# Autodesk Inventor assembly: CNC-FullAssembly
(part 2 of 3)
404. 91274A125-M5x8mm:5
405. 91274A125-M5x8mm:6
406. 91274A125-M5x8mm:7 — Mate:82, Mate:83
407. 91274A125-M5x8mm:8
408. 91274A125-M5x8mm:9
409. 91274A125-M5x8mm:13 — Mate:84, Mate:85
410. 91274A125-M5x8mm:14
411. 91274A125-M5x8mm:15
412. 91274A125-M5x8mm:16
413. 91274A125-M5x8mm:17
414. 91274A125-M5x8mm:18
415. 91274A125-M5x8mm:19 — Mate:86, Mate:87
416. 91274A125-M5x8mm:20
417. 91274A125-M5x8mm:21
418. 91290A231-M5x15mm:41 — Mate:226, Flush:128
419. 91290A231-M5x15mm:40 — Mate:224, Mate:225, Flush:128
420. 91290A231-M5x15mm:67
421. 91290A231-M5x15mm:68
422. 91290A231-M5x15mm:69
423. 91290A231-M5x15mm:70
424. 91290A231-M5x15mm:71
425. 91290A231-M5x15mm:72
426. 91290A231-M5x15mm:73
427. 91290A231-M5x15mm:74
428. 91290A231-M5x15mm:75
429. 91290A231-M5x15mm:76
430. 91290A231-M5x15mm:77
431. 91290A231-M5x15mm:78
432. 91290A231-M5x15mm:79
433. 91290A231-M5x15mm:80
434. 91290A231-M5x15mm:81 — Mate:314
435. 91290A231-M5x15mm:82 — Mate:313
436. 91290A231-M5x15mm:83 — Mate:292, Flush:148
437. 91290A231-M5x15mm:1 — Mate:288, Mate:289, Flush:148
438. 91290A231-M5x15mm:84
439. 91290A231-M5x15mm:85
440. 91290A231-M5x15mm:86
441. 91290A231-M5x15mm:87
442. 91290A231-M5x15mm:88
443. 91290A231-M5x15mm:89
444. 91290A231-M5x15mm:90
445. 91290A231-M5x15mm:91
446. 91290A231-M5x15mm:92
447. 91290A231-M5x15mm:93
448. 91290A231-M5x15mm:94
449. 91290A231-M5x15mm:95
450. 91290A231-M5x15mm:114 — Mate:595, Flush:298
451. 91290A231-M5x15mm:116
452. 91290A231-M5x15mm:117
453. 91290A231-M5x15mm:118
454. 91290A231-M5x15mm:115 — Mate:596, Flush:297, Flush:298
455. 91290A231-M5x15mm:119
456. 91290A231-M5x15mm:120
457. 91290A231-M5x15mm:121
458. 91290A231-M5x15mm:113 — Mate:597, Flush:296, Flush:297
459. 91290A231-M5x15mm:122
460. 91290A231-M5x15mm:123
461. 91290A231-M5x15mm:124
462. 91290A231-M5x15mm:112 — Mate:598, Mate:599, Flush:296
463. 91290A231-M5x15mm:125
464. 91290A231-M5x15mm:126
465. 91290A231-M5x15mm:127
466. 91290A231-M5x15mm:128 — Mate:622, Mate:623
467. 91290A231-M5x15mm:129
468. 91290A231-M5x15mm:130
## Component patterns: (4 elements, first: 91290A231-M5x15mm:20), (4 elements, first: 91290A231-M5x15mm:19), (6 elements, first: 91274A125-M5x8mm:1), (3 elements, first: 91274A125-M5x8mm:7), (6 elements, first: 91274A125-M5x8mm:13), (3 elements, first: 91274A125-M5x8mm:19), (9 elements, first: 91290A231-M5x15mm:41 + 91290A231-M5x15mm:40), (7 elements, first: 91290A231-M5x15mm:83 + 91290A231-M5x15mm:1), (4 elements, first: 91290A231-M5x15mm:114), (4 elements, first: 91290A231-M5x15mm:115), (4 elements, first: 91290A231-M5x15mm:113), (4 elements, first: 91290A231-M5x15mm:112), (3 elements, first: 91290A231-M5x15mm:128)
## Relationships (920: Mate 599, Flush 280, Angle 26, Tangent 14, Symmetry 1)
- Mate:1 (-20 mm): 40x40x500mm-Extrusion:1
- Mate:2 (-20 mm): 40x40x500mm-Extrusion:1
- Flush:1 (-250 mm): 40x40x500mm-Extrusion:1
- Flush:2: 40x40x500mm-Extrusion:1 ↔ 40x40x500mm-Extrusion:2
- Flush:3: 40x40x500mm-Extrusion:1 ↔ 40x40x500mm-Extrusion:2
- Mate:3: SFU1605-BallScrewNut:1 ↔ DSG16H-BallScrewFixtureBlock:1
- Mate:4: SFU1605-BallScrewNut:1 ↔ DSG16H-BallScrewFixtureBlock:1
- Mate:5: SFU1605-BallScrewNut:1 ↔ DSG16H-BallScrewFixtureBlock:1
- Angle:1 (0 deg): 40x40x500mm-Extrusion:1 ↔ DSG16H-BallScrewFixtureBlock:1
- Angle:2 (0 deg): 40x40x500mm-Extrusion:2 ↔ BK12-BallScrewStabilizer:1
- Flush:10: HGH20-LinearRailCarriage:1 ↔ HGH20-LinearRailCarriage:3
- Flush:11: HGH20-LinearRailCarriage:1 ↔ HGH20-LinearRailCarriage:4
- Mate:18 (40 mm): HGH20-LinearRailCarriage:1 ↔ HGH20-LinearRailCarriage:4
- Flush:12: HGH20-LinearRailCarriage:2 ↔ HGH20-LinearRailCarriage:3
- Flush:13: HGH20-LinearRailCarriage:2 ↔ HGH20-LinearRailCarriage:4
- Flush:14: DSG16H-BallScrewFixtureBlock:1 ↔ HGH20-LinearRailCarriage:1
- Mate:20: DSG16H-BallScrewFixtureBlock:1 ↔ HGH20-LinearRailCarriage:3
- Mate:21: SFU1605-BallScrewNut:1 ↔ 91274A131_M5x20mm:1
- Mate:22: SFU1605-BallScrewNut:1 ↔ 91274A131_M5x20mm:1
- Mate:23: SFU1605-BallScrewNut:1 ↔ 91274A131_M5x20mm:5
- Mate:24: SFU1605-BallScrewNut:1 ↔ 91274A131_M5x20mm:6
- Mate:25: SFU1605-BallScrewNut:1 ↔ 91274A131_M5x20mm:4
- Mate:26: SFU1605-BallScrewNut:1 ↔ 91274A131_M5x20mm:2
- Mate:27: SFU1605-BallScrewNut:1 ↔ 91274A131_M5x20mm:3
- Flush:15: 91274A131_M5x20mm:2 ↔ 91274A131_M5x20mm:3
- Flush:16: 91274A131_M5x20mm:2 ↔ 91274A131_M5x20mm:4
- Flush:17: 91274A131_M5x20mm:1 ↔ 91274A131_M5x20mm:4
- Flush:18: 91274A131_M5x20mm:1 ↔ 91274A131_M5x20mm:5
- Flush:19: 91274A131_M5x20mm:5 ↔ 91274A131_M5x20mm:6
- Mate:32: Nema23-StepperMotor:1 ↔ MH2025-6.35x10mmCoupler:1
- Angle:3 (0 deg): 40x40x500mm-Extrusion:1 ↔ Nema23-StepperMotor:1
- Mate:33 (2 mm): Nema23-StepperMotor:1 ↔ MH2025-6.35x10mmCoupler:1
- Angle:4 (0 deg): 40x40x500mm-Extrusion:1 ↔ BF12-BallScrewStabilizer2:1
- Mate:39: 40x40x500mm-Extrusion:2 ↔ CNC-000-StructureGusset1:1
- Mate:40: 40x40x500mm-Extrusion:2 ↔ CNC-000-StructureGusset1:1
- Mate:41: 40x40x500mm-Extrusion:2 ↔ CNC-000-StructureGusset1:1
- Mate:42: CNC-000-StructureGusset1:1 ↔ 91290A231-M5x15mm:19
- Mate:43: CNC-000-StructureGusset1:1 ↔ 91290A231-M5x15mm:19
- Mate:44: CNC-000-StructureGusset1:1 ↔ 91290A231-M5x15mm:20
- Mate:45: CNC-000-StructureGusset1:1 ↔ 91290A231-M5x15mm:20
- Flush:20: 40x40x500mm-Extrusion:1 ↔ 20x40x500mm-Extrusion:1
- Flush:21: 40x40x500mm-Extrusion:1 ↔ 20x40x500mm-Extrusion:1
- Flush:22: 40x40x500mm-Extrusion:2 ↔ 20x40x500mm-Extrusion:2
- Flush:23: 40x40x500mm-Extrusion:2 ↔ 20x40x500mm-Extrusion:2
- Mate:48: 40x40x500mm-Extrusion:1 ↔ CNC-001-StructureGusset2:1
- Mate:49: 40x40x500mm-Extrusion:1 ↔ CNC-001-StructureGusset2:1
- Mate:51: CNC-001-StructureGusset2:1 ↔ 91290A231-M5x15mm:27
- Mate:52: CNC-001-StructureGusset2:1 ↔ 91290A231-M5x15mm:27
- Mate:53: CNC-001-StructureGusset2:1 ↔ 91290A231-M5x15mm:30
- Mate:54: CNC-001-StructureGusset2:1 ↔ 91290A231-M5x15mm:28
- Mate:55: CNC-001-StructureGusset2:1 ↔ 91290A231-M5x15mm:29
- Flush:24: 91290A231-M5x15mm:28 ↔ 91290A231-M5x15mm:29
- Flush:25: 91290A231-M5x15mm:27 ↔ 91290A231-M5x15mm:28
- Flush:26: 91290A231-M5x15mm:27 ↔ 91290A231-M5x15mm:30
- Mate:56: BF12-BallScrewStabilizer2:1 ↔ CNC-002-ShimStructureGusset2:1
- Mate:57: BF12-BallScrewStabilizer2:1 ↔ CNC-002-ShimStructureGusset2:1
- Mate:58: BF12-BallScrewStabilizer2:1 ↔ CNC-002-ShimStructureGusset2:1
- Mate:59: Nema23-StepperMotor:1 ↔ 91274A131_M5x20mm:9
- Mate:60: Nema23-StepperMotor:1 ↔ 91274A131_M5x20mm:7
- Mate:61: Nema23-StepperMotor:1 ↔ 91274A131_M5x20mm:10
- Mate:62: Nema23-StepperMotor:1 ↔ 91274A131_M5x20mm:8
- Mate:63: Nema23-StepperMotor:1 ↔ 91274A131_M5x20mm:8
- Flush:27: 91274A131_M5x20mm:8 ↔ 91274A131_M5x20mm:10
- Flush:28: 91274A131_M5x20mm:9 ↔ 91274A131_M5x20mm:10
- Flush:29: 91274A131_M5x20mm:7 ↔ 91274A131_M5x20mm:9
- Mate:64: 91274A131_M5x20mm:9 ↔ 90576A104-M5-NylockNut:1
- Mate:65: CNC-000-StructureGusset1:1 ↔ 90576A104-M5-NylockNut:1
- Mate:66: 91274A131_M5x20mm:10 ↔ 90576A104-M5-NylockNut:2
- Mate:67: 91274A131_M5x20mm:7 ↔ 90576A104-M5-NylockNut:4
- Mate:68: 91274A131_M5x20mm:8 ↔ 90576A104-M5-NylockNut:3
- Flush:30: 90576A104-M5-NylockNut:2 ↔ 90576A104-M5-NylockNut:3
- Flush:31: 90576A104-M5-NylockNut:3 ↔ 90576A104-M5-NylockNut:4
- Flush:32: 90576A104-M5-NylockNut:1 ↔ 90576A104-M5-NylockNut:4
- Mate:75: 20x40x500mm-Extrusion:1 ↔ CNC-003-StructureGusset3:1
- Flush:35 (4.225 mm): 40x40x500mm-Extrusion:1 ↔ CNC-003-StructureGusset3:1
- Flush:36 (-4.225 mm): 20x40x500mm-Extrusion:1 ↔ CNC-003-StructureGusset3:1
- Mate:76: 20x40x500mm-Extrusion:2 ↔ CNC-003-StructureGusset3:2
- Flush:37 (-4.225 mm): 20x40x500mm-Extrusion:2 ↔ CNC-003-StructureGusset3:2
- Flush:38 (4.225 mm): 40x40x500mm-Extrusion:2 ↔ CNC-003-StructureGusset3:2
- Mate:77: CNC-000-StructureGusset1:1 ↔ CNC-004-Nema23Shim:1
- Mate:78: 90576A104-M5-NylockNut:2 ↔ CNC-004-Nema23Shim:1
- Mate:79: CNC-000-StructureGusset1:1 ↔ CNC-004-Nema23Shim:1
- Mate:80: CNC-003-StructureGusset3:1 ↔ 91274A125-M5x8mm:1
- Mate:81: CNC-003-StructureGusset3:1 ↔ 91274A125-M5x8mm:1
- Mate:82: CNC-003-StructureGusset3:1 ↔ 91274A125-M5x8mm:7
- Mate:83: CNC-003-StructureGusset3:1 ↔ 91274A125-M5x8mm:7
- Mate:84: CNC-003-StructureGusset3:2 ↔ 91274A125-M5x8mm:13
- Mate:85: CNC-003-StructureGusset3:2 ↔ 91274A125-M5x8mm:13
- Mate:86: CNC-003-StructureGusset3:2 ↔ 91274A125-M5x8mm:19
- Mate:87: CNC-003-StructureGusset3:2 ↔ 91274A125-M5x8mm:19
- Mate:91: HGH20-LinearRailCarriage:5 ↔ HGR20R-LinearRail500mm:4
- Mate:92: HGH20-LinearRailCarriage:5 ↔ HGR20R-LinearRail500mm:4
- Flush:50: HGR20R-LinearRail500mm:3 ↔ HGR20R-LinearRail500mm:4
- Angle:6 (180 deg): DSG16H-BallScrewFixtureBlock:1 ↔ DSG16H-BallScrewFixtureBlock:2
- Mate:94: DSG16H-BallScrewFixtureBlock:2 ↔ SFU1605-BallScrewNut:2
- Mate:95: DSG16H-BallScrewFixtureBlock:2 ↔ SFU1605-BallScrewNut:2
- Mate:96: DSG16H-BallScrewFixtureBlock:2 ↔ SFU1605-BallScrewNut:2
- Mate:97: DSG16H-BallScrewFixtureBlock:2 ↔ SFU1605-BallScrew500mm:2
- Mate:98: DSG16H-BallScrewFixtureBlock:1 ↔ CNC-005-XAxisMount1:1
- Mate:99: DSG16H-BallScrewFixtureBlock:1 ↔ CNC-005-XAxisMount1:1
- Mate:100: HGH20-LinearRailCarriage:1 ↔ CNC-005-XAxisMount1:1
- Mate:101: CNC-005-XAxisMount1:1 ↔ 91263A832-M5x10mm-Countersink:1
- Flush:53: CNC-005-XAxisMount1:1 ↔ 91263A832-M5x10mm-Countersink:1
- Mate:102: CNC-005-XAxisMount1:1 ↔ 91263A832-M5x10mm-Countersink:3
- Mate:103: CNC-005-XAxisMount1:1 ↔ 91263A832-M5x10mm-Countersink:4
- Mate:104: CNC-005-XAxisMount1:1 ↔ 91263A832-M5x10mm-Countersink:2
- Flush:54: 91263A832-M5x10mm-Countersink:3 ↔ 91263A832-M5x10mm-Countersink:4
- Flush:55: 91263A832-M5x10mm-Countersink:2 ↔ 91263A832-M5x10mm-Countersink:3
- Flush:56: 91263A832-M5x10mm-Countersink:1 ↔ 91263A832-M5x10mm-Countersink:3
- Mate:105: CNC-005-XAxisMount1:1 ↔ 91263A832-M5x10mm-Countersink:5
- Mate:106: CNC-005-XAxisMount1:1 ↔ 91263A832-M5x10mm-Countersink:6
- Mate:107: CNC-005-XAxisMount1:1 ↔ 91263A832-M5x10mm-Countersink:8
- Mate:108: CNC-005-XAxisMount1:1 ↔ 91263A832-M5x10mm-Countersink:7
- Flush:57: CNC-005-XAxisMount1:1 ↔ 91263A832-M5x10mm-Countersink:7
- Flush:58: CNC-005-XAxisMount1:1 ↔ 91263A832-M5x10mm-Countersink:6
- Flush:59: CNC-005-XAxisMount1:1 ↔ 91263A832-M5x10mm-Countersink:5
- Flush:60: CNC-005-XAxisMount1:1 ↔ 91263A832-M5x10mm-Countersink:8
- Mate:109: CNC-005-XAxisMount1:1 ↔ 91263A832-M5x10mm-Countersink:11
- Mate:110: CNC-005-XAxisMount1:1 ↔ 91263A832-M5x10mm-Countersink:12
- Mate:111: CNC-005-XAxisMount1:1 ↔ 91263A832-M5x10mm-Countersink:10
- Mate:112: CNC-005-XAxisMount1:1 ↔ 91263A832-M5x10mm-Countersink:9
- Flush:61: CNC-005-XAxisMount1:1 ↔ 91263A832-M5x10mm-Countersink:10
- Flush:62: 91263A832-M5x10mm-Countersink:9 ↔ 91263A832-M5x10mm-Countersink:10
- Flush:63: CNC-005-XAxisMount1:1 ↔ 91263A832-M5x10mm-Countersink:11
- Flush:64: 91263A832-M5x10mm-Countersink:11 ↔ 91263A832-M5x10mm-Countersink:12
- Mate:113: CNC-005-XAxisMount1:1 ↔ 91263A832-M5x10mm-Countersink:13
- Mate:114: CNC-005-XAxisMount1:1 ↔ 91263A832-M5x10mm-Countersink:16
- Mate:115: CNC-005-XAxisMount1:1 ↔ 91263A832-M5x10mm-Countersink:15
- Mate:116: CNC-005-XAxisMount1:1 ↔ 91263A832-M5x10mm-Countersink:14
- Flush:65: CNC-005-XAxisMount1:1 ↔ 91263A832-M5x10mm-Countersink:13
- Flush:66: CNC-005-XAxisMount1:1 ↔ 91263A832-M5x10mm-Countersink:15
- Flush:67: CNC-005-XAxisMount1:1 ↔ 91263A832-M5x10mm-Countersink:14
- Flush:68: CNC-005-XAxisMount1:1 ↔ 91263A832-M5x10mm-Countersink:16
- Mate:117: CNC-005-XAxisMount1:1 ↔ 91263A832-M5x10mm-Countersink:19
- Mate:118: CNC-005-XAxisMount1:1 ↔ 91263A832-M5x10mm-Countersink:17
- Mate:119: CNC-005-XAxisMount1:1 ↔ 91263A832-M5x10mm-Countersink:18
- Mate:120: CNC-005-XAxisMount1:1 ↔ 91263A832-M5x10mm-Countersink:20
- Flush:69: CNC-005-XAxisMount1:1 ↔ 91263A832-M5x10mm-Countersink:18
- Flush:70: CNC-005-XAxisMount1:1 ↔ 91263A832-M5x10mm-Countersink:20
- Flush:71: CNC-005-XAxisMount1:1 ↔ 91263A832-M5x10mm-Countersink:17
- Flush:72: CNC-005-XAxisMount1:1 ↔ 91263A832-M5x10mm-Countersink:19
- Mate:121: DSG16H-BallScrewFixtureBlock:2 ↔ CNC-006-XAxisMount2:1
- Mate:122: DSG16H-BallScrewFixtureBlock:2 ↔ CNC-006-XAxisMount2:1
- Mate:123: DSG16H-BallScrewFixtureBlock:2 ↔ CNC-006-XAxisMount2:1
- Mate:124: CNC-005-XAxisMount1:1 ↔ CNC-006-XAxisMount2:1
- Angle:7 (0 deg): CNC-005-XAxisMount1:1 ↔ CNC-006-XAxisMount2:1
- Mate:125: HGH20-LinearRailCarriage:7 ↔ CNC-006-XAxisMount2:1
- Mate:126: HGH20-LinearRailCarriage:7 ↔ CNC-006-XAxisMount2:1
- Mate:127: HGH20-LinearRailCarriage:7 ↔ CNC-006-XAxisMount2:1
- Mate:128: HGH20-LinearRailCarriage:6 ↔ CNC-006-XAxisMount2:1
- Mate:129: HGH20-LinearRailCarriage:6 ↔ CNC-006-XAxisMount2:1
- Mate:130: HGH20-LinearRailCarriage:6 ↔ CNC-006-XAxisMount2:1
- Mate:131: HGH20-LinearRailCarriage:5 ↔ CNC-006-XAxisMount2:1
- Mate:132: HGH20-LinearRailCarriage:5 ↔ CNC-006-XAxisMount2:1
- Mate:133: HGH20-LinearRailCarriage:5 ↔ CNC-006-XAxisMount2:1
- Mate:134: HGH20-LinearRailCarriage:8 ↔ CNC-006-XAxisMount2:1
- Mate:135: HGH20-LinearRailCarriage:8 ↔ CNC-006-XAxisMount2:1
- Mate:136: HGH20-LinearRailCarriage:8 ↔ CNC-006-XAxisMount2:1
- Mate:137: HGH20-LinearRailCarriage:8 ↔ HGR20R-LinearRail500mm:3
- Mate:138: HGH20-LinearRailCarriage:8 ↔ HGR20R-LinearRail500mm:3
- Mate:139: SFU1605-BallScrewNut:2 ↔ 91274A131_M5x20mm:11
- Mate:140: SFU1605-BallScrewNut:2 ↔ 91274A131_M5x20mm:11
- Mate:141: SFU1605-BallScrewNut:2 ↔ 91274A131_M5x20mm:14
- Mate:142: SFU1605-BallScrewNut:2 ↔ 91274A131_M5x20mm:16
- Mate:143: SFU1605-BallScrewNut:2 ↔ 91274A131_M5x20mm:15
- Mate:144: SFU1605-BallScrewNut:2 ↔ 91274A131_M5x20mm:13
- Mate:145: SFU1605-BallScrewNut:2 ↔ 91274A131_M5x20mm:12
- Flush:73: 91274A131_M5x20mm:14 ↔ 91274A131_M5x20mm:16
- Flush:74: 91274A131_M5x20mm:11 ↔ 91274A131_M5x20mm:14
- Flush:75: 91274A131_M5x20mm:11 ↔ 91274A131_M5x20mm:15
- Flush:76: 91274A131_M5x20mm:12 ↔ 91274A131_M5x20mm:16
- Flush:77: 91274A131_M5x20mm:12 ↔ 91274A131_M5x20mm:13
- Mate:146: CNC-006-XAxisMount2:1 ↔ 91263A832-M5x10mm-Countersink:22
- Mate:147: CNC-006-XAxisMount2:1 ↔ 91263A832-M5x10mm-Countersink:23
- Mate:148: CNC-006-XAxisMount2:1 ↔ 91263A832-M5x10mm-Countersink:24
- Mate:149: CNC-006-XAxisMount2:1 ↔ 91263A832-M5x10mm-Countersink:21
- Flush:78: CNC-006-XAxisMount2:1 ↔ 91263A832-M5x10mm-Countersink:21
- Flush:79: CNC-006-XAxisMount2:1 ↔ 91263A832-M5x10mm-Countersink:23
- Flush:80: 91263A832-M5x10mm-Countersink:22 ↔ 91263A832-M5x10mm-Countersink:23
- Flush:81: CNC-006-XAxisMount2:1 ↔ 91263A832-M5x10mm-Countersink:24
- Mate:150: CNC-006-XAxisMount2:1 ↔ 91263A832-M5x10mm-Countersink:25
- Mate:151: CNC-006-XAxisMount2:1 ↔ 91263A832-M5x10mm-Countersink:27
- Mate:152: CNC-006-XAxisMount2:1 ↔ 91263A832-M5x10mm-Countersink:28
- Mate:153: CNC-006-XAxisMount2:1 ↔ 91263A832-M5x10mm-Countersink:26
- Flush:82: CNC-006-XAxisMount2:1 ↔ 91263A832-M5x10mm-Countersink:27
- Flush:83: CNC-006-XAxisMount2:1 ↔ 91263A832-M5x10mm-Countersink:26
- Flush:84: CNC-006-XAxisMount2:1 ↔ 91263A832-M5x10mm-Countersink:28
- Flush:85: CNC-006-XAxisMount2:1 ↔ 91263A832-M5x10mm-Countersink:25
- Mate:154: CNC-006-XAxisMount2:1 ↔ 91263A832-M5x10mm-Countersink:31
- Mate:155: CNC-006-XAxisMount2:1 ↔ 91263A832-M5x10mm-Countersink:30
- Mate:156: CNC-006-XAxisMount2:1 ↔ 91263A832-M5x10mm-Countersink:29
- Mate:157: CNC-006-XAxisMount2:1 ↔ 91263A832-M5x10mm-Countersink:32
- Flush:86: CNC-006-XAxisMount2:1 ↔ 91263A832-M5x10mm-Countersink:32
- Flush:87: CNC-006-XAxisMount2:1 ↔ 91263A832-M5x10mm-Countersink:29
- Flush:88: 91263A832-M5x10mm-Countersink:29 ↔ 91263A832-M5x10mm-Countersink:31
- Flush:89: 91263A832-M5x10mm-Countersink:30 ↔ 91263A832-M5x10mm-Countersink:31
- Mate:158: CNC-006-XAxisMount2:1 ↔ 91263A832-M5x10mm-Countersink:35
- Mate:159: CNC-006-XAxisMount2:1 ↔ 91263A832-M5x10mm-Countersink:33
- Mate:160: CNC-006-XAxisMount2:1 ↔ 91263A832-M5x10mm-Countersink:34
- Mate:161: CNC-006-XAxisMount2:1 ↔ 91263A832-M5x10mm-Countersink:36
- Flush:90: CNC-006-XAxisMount2:1 ↔ 91263A832-M5x10mm-Countersink:36
- Flush:91: CNC-006-XAxisMount2:1 ↔ 91263A832-M5x10mm-Countersink:34
- Flush:92: CNC-006-XAxisMount2:1 ↔ 91263A832-M5x10mm-Countersink:35
- Flush:93: CNC-006-XAxisMount2:1 ↔ 91263A832-M5x10mm-Countersink:33
- Mate:162: CNC-006-XAxisMount2:1 ↔ 91263A832-M5x10mm-Countersink:38
- Mate:163: CNC-006-XAxisMount2:1 ↔ 91263A832-M5x10mm-Countersink:39
- Mate:164: CNC-006-XAxisMount2:1 ↔ 91263A832-M5x10mm-Countersink:37
- Mate:165: CNC-006-XAxisMount2:1 ↔ 91263A832-M5x10mm-Countersink:40
- Flush:94: CNC-006-XAxisMount2:1 ↔ 91263A832-M5x10mm-Countersink:40
- Flush:95: CNC-006-XAxisMount2:1 ↔ 91263A832-M5x10mm-Countersink:37
- Flush:96: CNC-006-XAxisMount2:1 ↔ 91263A832-M5x10mm-Countersink:38
- Flush:97: CNC-006-XAxisMount2:1 ↔ 91263A832-M5x10mm-Countersink:39
- Mate:166: CNC-005-XAxisMount1:1 ↔ CNC-006-XAxisMount2:1
- Mate:167: CNC-006-XAxisMount2:1 ↔ 92095A495-M8-18mm-ButtonHead:1
- Mate:168: CNC-006-XAxisMount2:1 ↔ 92095A495-M8-18mm-ButtonHead:2
- Mate:169: CNC-006-XAxisMount2:1 ↔ 92095A495-M8-18mm-ButtonHead:3
- Mate:170: CNC-006-XAxisMount2:1 ↔ 92095A495-M8-18mm-ButtonHead:3
- Flush:98: 92095A495-M8-18mm-ButtonHead:1 ↔ 92095A495-M8-18mm-ButtonHead:3
- Flush:99: 92095A495-M8-18mm-ButtonHead:1 ↔ 92095A495-M8-18mm-ButtonHead:2
- Mate:171: CNC-006-XAxisMount2:1 ↔ 92095A495-M8-18mm-ButtonHead:8
- Flush:100: 92095A495-M8-18mm-ButtonHead:3 ↔ 92095A495-M8-18mm-ButtonHead:8
- Mate:172: CNC-006-XAxisMount2:1 ↔ 92095A495-M8-18mm-ButtonHead:11
- Mate:173: CNC-006-XAxisMount2:1 ↔ 92095A495-M8-18mm-ButtonHead:12
- Flush:101: 92095A495-M8-18mm-ButtonHead:11 ↔ 92095A495-M8-18mm-ButtonHead:12
- Flush:102: 92095A495-M8-18mm-ButtonHead:1 ↔ 92095A495-M8-18mm-ButtonHead:11
- Mate:174: CNC-006-XAxisMount2:1 ↔ 92095A495-M8-18mm-ButtonHead:9
- Mate:175: CNC-006-XAxisMount2:1 ↔ 92095A495-M8-18mm-ButtonHead:10
- Flush:103: 92095A495-M8-18mm-ButtonHead:9 ↔ 92095A495-M8-18mm-ButtonHead:10
- Flush:104: 92095A495-M8-18mm-ButtonHead:2 ↔ 92095A495-M8-18mm-ButtonHead:9
- Mate:176: 92095A495-M8-18mm-ButtonHead:1 ↔ 94645A210-M8-NylockNut:1
- Mate:177: CNC-005-XAxisMount1:1 ↔ 94645A210-M8-NylockNut:1
- Mate:178: 92095A495-M8-18mm-ButtonHead:2 ↔ 94645A210-M8-NylockNut:2
- Mate:179: CNC-005-XAxisMount1:1 ↔ 94645A210-M8-NylockNut:2
- Mate:180: 92095A495-M8-18mm-ButtonHead:3 ↔ 94645A210-M8-NylockNut:3
- Mate:181: CNC-005-XAxisMount1:1 ↔ 94645A210-M8-NylockNut:3
- Mate:182: 92095A495-M8-18mm-ButtonHead:8 ↔ 94645A210-M8-NylockNut:4
- Mate:183: CNC-005-XAxisMount1:1 ↔ 94645A210-M8-NylockNut:4
- Mate:184: 92095A495-M8-18mm-ButtonHead:11 ↔ 94645A210-M8-NylockNut:5
- Mate:185: 92095A495-M8-18mm-ButtonHead:12 ↔ 94645A210-M8-NylockNut:6
- Mate:186: CNC-005-XAxisMount1:1 ↔ 94645A210-M8-NylockNut:6
- Mate:187: CNC-005-XAxisMount1:1 ↔ 94645A210-M8-NylockNut:5
- Mate:188: 92095A495-M8-18mm-ButtonHead:9 ↔ 94645A210-M8-NylockNut:7
- Mate:189: 92095A495-M8-18mm-ButtonHead:10 ↔ 94645A210-M8-NylockNut:8
- Mate:190: CNC-005-XAxisMount1:1 ↔ 94645A210-M8-NylockNut:8
- Mate:191: CNC-005-XAxisMount1:1 ↔ 94645A210-M8-NylockNut:7
- Flush:106: HGR20R-LinearRail500mm:4 ↔ 20x40x500mm-Extrusion2:1
- Flush:107: HGR20R-LinearRail500mm:4 ↔ 20x40x500mm-Extrusion2:1
- Flush:108: 20x40x500mm-Extrusion2:1 ↔ 20x40x500mm-Extrusion2:2
- Mate:193: 20x40x500mm-Extrusion2:1 ↔ 20x40x500mm-Extrusion2:2
- Flush:109: 20x40x500mm-Extrusion2:1 ↔ 20x40x500mm-Extrusion2:2
- Flush:110: 20x40x500mm-Extrusion2:2 ↔ 20x40x500mm-Extrusion2:3
- Flush:111: 20x40x500mm-Extrusion2:2 ↔ 20x40x500mm-Extrusion2:3
- Mate:194: 20x40x500mm-Extrusion2:2 ↔ 20x40x500mm-Extrusion2:3
- Flush:116: 20x40x500mm-Extrusion2:1 ↔ 20x20x500mm_Extrusion:3
- Mate:199: HGR20R-LinearRail500mm:4 ↔ 20x20x500mm_Extrusion:3
- Flush:117: 20x40x500mm-Extrusion2:1 ↔ 20x20x500mm_Extrusion:3
- Mate:200: 20x40x500mm-Extrusion2:1 ↔ 20x20x500mm_Extrusion:3
- Mate:201: 20x40x500mm-Extrusion2:3 ↔ 20x40x500mm-Extrusion2:4
- Flush:118: 20x40x500mm-Extrusion2:3 ↔ 20x40x500mm-Extrusion2:4
- Mate:202: HGR20R-LinearRail500mm:3 ↔ 20x40x500mm-Extrusion2:4
- Mate:203: SFU1605-BallScrew500mm:2 ↔ BF12-BallScrewStabilizer2:2
- Mate:204: SFU1605-BallScrew500mm:2 ↔ BF12-BallScrewStabilizer2:2
- Flush:119: HGR20R-LinearRail500mm:4 ↔ BF12-BallScrewStabilizer2:2
- Angle:8 (0 deg): 20x40x500mm-Extrusion2:2 ↔ BF12-BallScrewStabilizer2:2
- Mate:205: SFU1605-BallScrew500mm:2 ↔ Nema23-StepperMotor:2
- Angle:9 (0 deg): 20x40x500mm-Extrusion2:2 ↔ Nema23-StepperMotor:2
- Mate:206: Nema23-StepperMotor:2 ↔ MH2025-6.35x10mmCoupler:2
- Mate:207 (2 mm): SFU1605-BallScrew500mm:2 ↔ MH2025-6.35x10mmCoupler:2
- Mate:208 (2 mm): Nema23-StepperMotor:2 ↔ MH2025-6.35x10mmCoupler:2
- Mate:209: SFU1605-BallScrew500mm:2 ↔ BK12-BallScrewStabilizer:2
- Angle:10 (0 deg): HGR20R-LinearRail500mm:4 ↔ BK12-BallScrewStabilizer:2
- Mate:211: 20x40x500mm-Extrusion2:1 ↔ CNC-007-XAxisBallScrewMount:1
- Mate:212: 20x40x500mm-Extrusion2:1 ↔ CNC-007-XAxisBallScrewMount:1
- Mate:213: 20x40x500mm-Extrusion2:1 ↔ CNC-007-XAxisBallScrewMount:1
- Mate:214: CNC-007-XAxisBallScrewMount:1 ↔ 91290A231-M5x15mm:36
- Mate:215: CNC-007-XAxisBallScrewMount:1 ↔ 91290A231-M5x15mm:33
- Mate:216: CNC-007-XAxisBallScrewMount:1 ↔ 91290A231-M5x15mm:34
- Mate:217: CNC-007-XAxisBallScrewMount:1 ↔ 91290A231-M5x15mm:37
- Mate:218: CNC-007-XAxisBallScrewMount:1 ↔ 91290A231-M5x15mm:32
- Mate:219: CNC-007-XAxisBallScrewMount:1 ↔ 91290A231-M5x15mm:31
- Mate:220: CNC-007-XAxisBallScrewMount:1 ↔ 91290A231-M5x15mm:35
- Mate:221: CNC-007-XAxisBallScrewMount:1 ↔ 91290A231-M5x15mm:36
- Flush:120: 91290A231-M5x15mm:33 ↔ 91290A231-M5x15mm:34
- Flush:121: 91290A231-M5x15mm:33 ↔ 91290A231-M5x15mm:37
- Flush:122: 91290A231-M5x15mm:32 ↔ 91290A231-M5x15mm:37
- Flush:123: 91290A231-M5x15mm:31 ↔ 91290A231-M5x15mm:32
- Flush:124: 91290A231-M5x15mm:31 ↔ 91290A231-M5x15mm:35
- Flush:125: 91290A231-M5x15mm:32 ↔ 91290A231-M5x15mm:36
- Mate:222: CNC-007-XAxisBallScrewMount:1 ↔ 91290A231-M5x15mm:38
- Flush:126: 91290A231-M5x15mm:36 ↔ 91290A231-M5x15mm:38
- Mate:223: CNC-007-XAxisBallScrewMount:1 ↔ 91290A231-M5x15mm:39
- Flush:127: 91290A231-M5x15mm:32 ↔ 91290A231-M5x15mm:39
- Mate:224: HGR20R-LinearRail500mm:4 ↔ 91290A231-M5x15mm:40
- Mate:225: HGR20R-LinearRail500mm:4 ↔ 91290A231-M5x15mm:40
- Mate:226: HGR20R-LinearRail500mm:3 ↔ 91290A231-M5x15mm:41
- Flush:128: 91290A231-M5x15mm:41 ↔ 91290A231-M5x15mm:40
- Mate:227: 20x40x500mm-Extrusion2:4 ↔ CNC-008-XAxisNema23Mount:1
- Mate:228: 20x40x500mm-Extrusion2:3 ↔ CNC-008-XAxisNema23Mount:1
- Mate:229: 20x40x500mm-Extrusion2:3 ↔ CNC-008-XAxisNema23Mount:1
- Mate:230: CNC-008-XAxisNema23Mount:1 ↔ 91290A231-M5x15mm:64
- Mate:231: CNC-008-XAxisNema23Mount:1 ↔ 91290A231-M5x15mm:59
- Mate:232: CNC-008-XAxisNema23Mount:1 ↔ 91290A231-M5x15mm:60
- Mate:233: CNC-008-XAxisNema23Mount:1 ↔ 91290A231-M5x15mm:58
- Mate:234: CNC-008-XAxisNema23Mount:1 ↔ 91290A231-M5x15mm:61
- Mate:235: CNC-008-XAxisNema23Mount:1 ↔ 91290A231-M5x15mm:62
- Mate:236: CNC-008-XAxisNema23Mount:1 ↔ 91290A231-M5x15mm:66
- Mate:237: CNC-008-XAxisNema23Mount:1 ↔ 91290A231-M5x15mm:65
- Mate:238: CNC-008-XAxisNema23Mount:1 ↔ 91290A231-M5x15mm:63
- Mate:239: CNC-008-XAxisNema23Mount:1 ↔ 91290A231-M5x15mm:63
- Flush:129: 91290A231-M5x15mm:63 ↔ 91290A231-M5x15mm:65
- Flush:130: 91290A231-M5x15mm:65 ↔ 91290A231-M5x15mm:66
- Flush:131: 91290A231-M5x15mm:62 ↔ 91290A231-M5x15mm:66
- Flush:132: 91290A231-M5x15mm:61 ↔ 91290A231-M5x15mm:62
- Flush:133: 91290A231-M5x15mm:58 ↔ 91290A231-M5x15mm:61
- Flush:134: 91290A231-M5x15mm:58 ↔ 91290A231-M5x15mm:59
- Flush:135: 91290A231-M5x15mm:59 ↔ 91290A231-M5x15mm:64
- Flush:136: 91290A231-M5x15mm:60 ↔ 91290A231-M5x15mm:64
- Mate:240: MH2025-6.35x10mmCoupler:2 ↔ CNC-009-XAxisNema23Spacer:1
- Mate:241: CNC-008-XAxisNema23Mount:1 ↔ CNC-009-XAxisNema23Spacer:1
- Mate:242: CNC-008-XAxisNema23Mount:1 ↔ CNC-009-XAxisNema23Spacer:1
- Mate:243: Nema23-StepperMotor:2 ↔ 91290A198-M5-50mm:2
- Mate:244: Nema23-StepperMotor:2 ↔ 91290A198-M5-50mm:1
- Mate:245: Nema23-StepperMotor:2 ↔ 91290A198-M5-50mm:3
- Mate:246: Nema23-StepperMotor:2 ↔ 91290A198-M5-50mm:4
- Mate:247: Nema23-StepperMotor:2 ↔ 91290A198-M5-50mm:4
- Flush:137: 91290A198-M5-50mm:3 ↔ 91290A198-M5-50mm:4
- Flush:138: 91290A198-M5-50mm:1 ↔ 91290A198-M5-50mm:2
- Flush:139: 91290A198-M5-50mm:2 ↔ 91290A198-M5-50mm:3
- Mate:248: 91290A198-M5-50mm:1 ↔ 90576A104-M5-NylockNut:6
- Mate:249: 91290A198-M5-50mm:4 ↔ 90576A104-M5-NylockNut:8
- Mate:250: 91290A198-M5-50mm:2 ↔ 90576A104-M5-NylockNut:7
- Mate:251: 91290A198-M5-50mm:3 ↔ 90576A104-M5-NylockNut:5
- Mate:252: CNC-008-XAxisNema23Mount:1 ↔ 90576A104-M5-NylockNut:5
- Mate:253: CNC-008-XAxisNema23Mount:1 ↔ 90576A104-M5-NylockNut:8
- Mate:254: CNC-008-XAxisNema23Mount:1 ↔ 90576A104-M5-NylockNut:6
- Mate:255: CNC-008-XAxisNema23Mount:1 ↔ 90576A104-M5-NylockNut:7
- Mate:256: SFU1605-BallScrew500mm:2 ↔ BK12-BallScrewStabilizer:2
- Angle:11 (0 deg): 20x40x500mm-Extrusion2:1 ↔ 3103-0001-0002-GobildaLimitSwitch:1
- Tangent:2: 20x40x500mm-Extrusion2:1 ↔ CNC-010-XAxisLimitSwitchMount:1
- Mate:258: 3103-0001-0002-GobildaLimitSwitch:1 ↔ CNC-010-XAxisLimitSwitchMount:1
- Mate:259: 3103-0001-0002-GobildaLimitSwitch:1 ↔ CNC-010-XAxisLimitSwitchMount:1
- Mate:264: 40x40x500mm-Extrusion:1 ↔ 91290A231-M5x15mm:22
- Mate:265: CNC-000-StructureGusset1:1 ↔ 90576A104-M5-NylockNut:2
- Mate:269: BF12-BallScrewStabilizer2:1 ↔ CNC-001-StructureGusset2:1
- Flush:142: HGH20-LinearRailCarriage:5 ↔ HGR20R-LinearRail500mm:4
- Tangent:3: 20x20x500mm_Extrusion:3 ↔ CNC-010-XAxisLimitSwitchMount:1
- Flush:143 (-1 mm): 20x40x500mm-Extrusion2:1 ↔ CNC-010-XAxisLimitSwitchMount:1
- Tangent:4: 20x40x500mm-Extrusion2:1 ↔ CNC-011-XAxisHardStop:1
- Tangent:5: 20x20x500mm_Extrusion:3 ↔ CNC-011-XAxisHardStop:1
- Mate:270: 20x40x500mm-Extrusion2:1 ↔ CNC-011-XAxisHardStop:1
- Flush:144 (21.565 mm): 20x20x500mm_Extrusion:3 ↔ CNC-011-XAxisHardStop:1
- Mate:271: CNC-011-XAxisHardStop:1 ↔ 91274A125-M5x8mm:25
- Mate:272: CNC-011-XAxisHardStop:1 ↔ 91274A125-M5x8mm:25
- Mate:273: CNC-011-XAxisHardStop:1 ↔ 91274A125-M5x8mm:26
- Flush:145: 91274A125-M5x8mm:25 ↔ 91274A125-M5x8mm:26
- Mate:274: CNC-011-XAxisHardStop:1 ↔ CNC-011-XAxisHardStop:2
- Mate:275: 91274A125-M5x8mm:26 ↔ CNC-011-XAxisHardStop:2
- Mate:276: 20x40x500mm-Extrusion2:4 ↔ CNC-011-XAxisHardStop:2
- Mate:277: CNC-011-XAxisHardStop:2 ↔ 91274A125-M5x8mm:27
- Mate:278: CNC-011-XAxisHardStop:2 ↔ 91274A125-M5x8mm:28
- Mate:279: CNC-011-XAxisHardStop:2 ↔ 91274A125-M5x8mm:28
- Mate:280: CNC-011-XAxisHardStop:2 ↔ 91274A125-M5x8mm:27
- Mate:281: HGH20-LinearRailCarriage:3 ↔ 91263A832-M5x10mm-Countersink:2
- Mate:282: HGH20-LinearRailCarriage:3 ↔ CNC-005-XAxisMount1:1
- Mate:283: HGH20-LinearRailCarriage:2 ↔ CNC-005-XAxisMount1:1
- Mate:284: HGH20-LinearRailCarriage:1 ↔ 91263A832-M5x10mm-Countersink:6
- Mate:285: HGH20-LinearRailCarriage:4 ↔ CNC-005-XAxisMount1:1
- Mate:286: 40x40x500mm-Extrusion:1 ↔ HGR20R-LinearRail300mm:2
- Flush:146: 40x40x500mm-Extrusion:1 ↔ HGR20R-LinearRail300mm:2
- Mate:287: CNC-000-StructureGusset1:1 ↔ HGR20R-LinearRail300mm:2
- Mate:288: HGR20R-LinearRail300mm:2 ↔ 91290A231-M5x15mm:1
- Mate:289: HGR20R-LinearRail300mm:2 ↔ 91290A231-M5x15mm:1
- Mate:290: 40x40x500mm-Extrusion:2 ↔ HGR20R-LinearRail300mm:1
- Mate:291: CNC-000-StructureGusset1:1 ↔ HGR20R-LinearRail300mm:1
- Flush:147: 40x40x500mm-Extrusion:2 ↔ HGR20R-LinearRail300mm:1
- Mate:292: HGR20R-LinearRail300mm:1 ↔ 91290A231-M5x15mm:83
- Flush:148: 91290A231-M5x15mm:83 ↔ 91290A231-M5x15mm:1
- Mate:293: 40x40x500mm-Extrusion:1 ↔ 20x40x500mm-Extrusion:1
- Mate:294: 40x40x500mm-Extrusion:2 ↔ 20x40x500mm-Extrusion:2
- Mate:295: BK12-BallScrewStabilizer:1 ↔ SFU1605-BallScrew400mm:1
- Mate:296: BK12-BallScrewStabilizer:1 ↔ SFU1605-BallScrew400mm:1
- Mate:297: MH2025-6.35x10mmCoupler:1 ↔ SFU1605-BallScrew400mm:1
- Mate:298: BF12-BallScrewStabilizer2:1 ↔ SFU1605-BallScrew400mm:1
- Mate:299: 40x40x500mm-Extrusion:2 ↔ CNC-001-StructureGusset2:1
- Mate:300: CNC-001-StructureGusset2:1 ↔ CNC-002-ShimStructureGusset2:1
- Mate:301: Nema23-StepperMotor:1 ↔ CNC-004-Nema23Shim:1
- Mate:302: CNC-000-StructureGusset1:1 ↔ 91290A231-M5x15mm:23
- Mate:303: HGH20-LinearRailCarriage:1 ↔ HGR20R-LinearRail300mm:2
- Mate:304: HGH20-LinearRailCarriage:1 ↔ HGR20R-LinearRail300mm:2
- Tangent:7 (78.25 mm): 40x40x500mm-Extrusion:1 ↔ RouterSpindle-65mm:1
- Tangent:8 (181.8503 mm): 20x40x500mm-Extrusion:1 ↔ RouterSpindle-65mm:1
- Mate:305: 3103-0001-0002-GobildaLimitSwitch:1 ↔ 90128A046-#2-.375in:1
- Mate:306: 3103-0001-0002-GobildaLimitSwitch:1 ↔ 90128A046-#2-.375in:2
- Mate:307: CNC-010-XAxisLimitSwitchMount:1 ↔ 90128A046-#2-.375in:2
- Mate:308: CNC-010-XAxisLimitSwitchMount:1 ↔ 90128A046-#2-.375in:1
- Mate:309: 90128A046-#2-.375in:2 ↔ 90480A003-#2-HexNut:1
- Mate:310: 3103-0001-0002-GobildaLimitSwitch:1 ↔ 90480A003-#2-HexNut:1
- Mate:311: 90128A046-#2-.375in:1 ↔ 90480A003-#2-HexNut:2
- Flush:149: 90480A003-#2-HexNut:1 ↔ 90480A003-#2-HexNut:2
- Mate:312: 20x20x500mm_Extrusion:3 ↔ CNC-010-XAxisLimitSwitchMount:1
- Mate:313: HGR20R-LinearRail500mm:4 ↔ 91290A231-M5x15mm:82
- Mate:314: HGR20R-LinearRail500mm:3 ↔ 91290A231-M5x15mm:81
- Mate:329: HGH20-LinearRailCarriage:2 ↔ 20x40x500mm-Extrusion:2
- Mate:330: 20x40x500mm-Extrusion:2 ↔ 20x40x100mm-Extrusion:3
- Flush:154: 20x40x500mm-Extrusion:2 ↔ 20x40x100mm-Extrusion:3
- Flush:155: 20x40x500mm-Extrusion:2 ↔ 20x40x100mm-Extrusion:3
- Flush:156: 20x40x500mm-Extrusion:1 ↔ 20x40x100mm-Extrusion:4
- Flush:157: 20x40x500mm-Extrusion:1 ↔ 20x40x100mm-Extrusion:4
- Mate:331: 20x40x500mm-Extrusion:1 ↔ 20x40x100mm-Extrusion:4
- Mate:336: 20x40x100mm-Extrusion:3 ↔ 20x40x128mm-Extrusion:1
- Flush:160: 20x40x100mm-Extrusion:3 ↔ 20x40x128mm-Extrusion:1
- Flush:161: 20x40x100mm-Extrusion:3 ↔ 20x40x128mm-Extrusion:1
- Flush:165: 91274A125-M5x8mm:29 ↔ 91274A125-M5x8mm:30
- Mate:349 (4.7625 mm): 20x40x128mm-Extrusion:1 ↔ HGH20-LinearRailCarriage:9
- Mate:352: 20x40x500mm-Extrusion:2 ↔ CNC-013-ZAxisMainMount:2
- Tangent:9: 20x40x500mm-Extrusion:2 ↔ CNC-013-ZAxisMainMount:2
- Tangent:10: 20x40x100mm-Extrusion:3 ↔ CNC-013-ZAxisMainMount:2
- Angle:17 (0 deg): 20x40x100mm-Extrusion:3 ↔ CNC-013-ZAxisMainMount:2
- Mate:353: CNC-013-ZAxisMainMount:1 ↔ CNC-013-ZAxisMainMount:2
- Mate:354: CNC-013-ZAxisMainMount:1 ↔ CNC-013-ZAxisMainMount:2
- Mate:355: 20x40x100mm-Extrusion:4 ↔ CNC-013-ZAxisMainMount:1
- Mate:356: 91274A125-M5x8mm:29 ↔ CNC-013-ZAxisMainMount:1
- Mate:357: 91274A125-M5x8mm:30 ↔ CNC-013-ZAxisMainMount:1
- Mate:358: 91274A125-M5x8mm:30 ↔ CNC-013-ZAxisMainMount:1
- Mate:359: CNC-013-ZAxisMainMount:1 ↔ 91274A125-M5x8mm:33
- Mate:360: CNC-013-ZAxisMainMount:1 ↔ 91274A125-M5x8mm:34
- Mate:361: CNC-013-ZAxisMainMount:1 ↔ 91274A125-M5x8mm:36
- Mate:362: CNC-013-ZAxisMainMount:1 ↔ 91274A125-M5x8mm:35
- Flush:169: 91274A125-M5x8mm:35 ↔ 91274A125-M5x8mm:36
- Flush:170: 91274A125-M5x8mm:29 ↔ 91274A125-M5x8mm:36
- Flush:171: 91274A125-M5x8mm:29 ↔ 91274A125-M5x8mm:34
- Flush:172: 91274A125-M5x8mm:29 ↔ 91274A125-M5x8mm:33
- Mate:363: 91274A125-M5x8mm:31 ↔ CNC-013-ZAxisMainMount:2
- Mate:364: 91274A125-M5x8mm:32 ↔ CNC-013-ZAxisMainMount:2
- Mate:365: 91274A125-M5x8mm:32 ↔ CNC-013-ZAxisMainMount:2
- Flush:173: 91274A125-M5x8mm:31 ↔ 91274A125-M5x8mm:32
- Mate:366: CNC-013-ZAxisMainMount:2 ↔ 91274A125-M5x8mm:37
- Mate:367: CNC-013-ZAxisMainMount:2 ↔ 91274A125-M5x8mm:40
- Mate:368: CNC-013-ZAxisMainMount:2 ↔ 91274A125-M5x8mm:39
- Mate:369: CNC-013-ZAxisMainMount:2 ↔ 91274A125-M5x8mm:38
- Flush:174: 91274A125-M5x8mm:38 ↔ 91274A125-M5x8mm:39
- Flush:175: 91274A125-M5x8mm:31 ↔ 91274A125-M5x8mm:38
- Flush:176: 91274A125-M5x8mm:31 ↔ 91274A125-M5x8mm:37
- Mate:370: CNC-013-ZAxisMainMount:1 ↔ 91274A134-M5x30mm:3
- Mate:371: CNC-013-ZAxisMainMount:1 ↔ 91274A134-M5x30mm:4
- Mate:372: CNC-013-ZAxisMainMount:1 ↔ 91274A134-M5x30mm:4
- Flush:177: 91274A134-M5x30mm:3 ↔ 91274A134-M5x30mm:4
- Mate:373: CNC-013-ZAxisMainMount:2 ↔ 91274A134-M5x30mm:1
- Mate:374: CNC-013-ZAxisMainMount:2 ↔ 91274A134-M5x30mm:2
- Mate:375: CNC-013-ZAxisMainMount:2 ↔ 91274A134-M5x30mm:2
- Flush:178: 91274A134-M5x30mm:1 ↔ 91274A134-M5x30mm:2
- Flush:180: HGH20-LinearRailCarriage:9 ↔ HGH20-LinearRailCarriage:10
- Flush:181: HGH20-LinearRailCarriage:9 ↔ HGH20-LinearRailCarriage:10
- Angle:18 (0 deg): HGH20-LinearRailCarriage:9 ↔ DSG16H-BallScrewFixtureBlock:3
- Flush:185: 20x40x100mm-Extrusion:3 ↔ HGH20-LinearRailCarriage:9
- Flush:186: 20x40x100mm-Extrusion:4 ↔ HGH20-LinearRailCarriage:10
- Mate:376: DSG16H-BallScrewFixtureBlock:3 ↔ BF12-BallScrewStabilizer2:3
- Angle:19 (0 deg): 20x40x128mm-Extrusion:1 ↔ DSG16H-BallScrewFixtureBlock:3
- Mate:378: 20x40x128mm-Extrusion:1 ↔ DSG16H-BallScrewFixtureBlock:3
- Mate:379: BF12-BallScrewStabilizer2:3 ↔ 92981A790-M5x40mm-ShoulderBolt:2
- Mate:380: BF12-BallScrewStabilizer2:3 ↔ 92981A790-M5x40mm-ShoulderBolt:1
- Mate:381: BF12-BallScrewStabilizer2:3 ↔ 92981A790-M5x40mm-ShoulderBolt:1
- Mate:382: BF12-BallScrewStabilizer2:3 ↔ 92981A790-M5x40mm-ShoulderBolt:2
- Mate:383: HGH20-LinearRailCarriage:9 ↔ HGR20R-LinearRail200mm:1
- Mate:384: HGH20-LinearRailCarriage:9 ↔ HGR20R-LinearRail200mm:1
- Mate:385: HGH20-LinearRailCarriage:10 ↔ HGR20R-LinearRail200mm:2
- Mate:386: HGH20-LinearRailCarriage:10 ↔ HGR20R-LinearRail200mm:2
- Flush:189: HGR20R-LinearRail200mm:1 ↔ HGR20R-LinearRail200mm:2
- Flush:191 (10 mm): RouterSpindle-65mm:1 ↔ HGR20R-LinearRail200mm:1
- Mate:387: 20x40x100mm-Extrusion:3 ↔ HGH20-LinearRailCarriage:9
- Mate:388: DSG16H-BallScrewFixtureBlock:3 ↔ SFU1605-BallScrewNut:3
- Mate:389: DSG16H-BallScrewFixtureBlock:3 ↔ SFU1605-BallScrewNut:3
- Mate:390: DSG16H-BallScrewFixtureBlock:3 ↔ SFU1605-BallScrewNut:3
- Mate:391: SFU1605-BallScrewNut:3 ↔ 91274A131_M5x20mm:18
- Mate:392: SFU1605-BallScrewNut:3 ↔ 91274A131_M5x20mm:17
- Mate:393: SFU1605-BallScrewNut:3 ↔ 91274A131_M5x20mm:19
- Mate:394: SFU1605-BallScrewNut:3 ↔ 91274A131_M5x20mm:22
- Mate:395: SFU1605-BallScrewNut:3 ↔ 91274A131_M5x20mm:20
- Mate:396: SFU1605-BallScrewNut:3 ↔ 91274A131_M5x20mm:21
- Mate:397: SFU1605-BallScrewNut:3 ↔ 91274A131_M5x20mm:18
- Flush:193: 91274A131_M5x20mm:17 ↔ 91274A131_M5x20mm:19
- Flush:194: 91274A131_M5x20mm:19 ↔ 91274A131_M5x20mm:22
- Flush:195: 91274A131_M5x20mm:20 ↔ 91274A131_M5x20mm:22
- Flush:196: 91274A131_M5x20mm:20 ↔ 91274A131_M5x20mm:21
- Flush:197: 91274A131_M5x20mm:18 ↔ 91274A131_M5x20mm:22
- Flush:198: HGH20-LinearRailCarriage:10 ↔ DSG16H-BallScrewFixtureBlock:3
- Flush:199: BF12-BallScrewStabilizer2:3 ↔ HGR20R-LinearRail200mm:2
- Angle:20 (0 deg): BF12-BallScrewStabilizer2:3 ↔ HGR20R-LinearRail200mm:2
- Mate:399: BF12-BallScrewStabilizer2:3 ↔ BK12-BallScrewStabilizer:3
- Angle:21 (0 deg): BF12-BallScrewStabilizer2:3 ↔ BK12-BallScrewStabilizer:3
- Mate:401: BK12-BallScrewStabilizer:3 ↔ MH2025-6.35x10mmCoupler:3
- Mate:402: Nema23-StepperMotor:3 ↔ MH2025-6.35x10mmCoupler:3
- Angle:22 (0 deg): BK12-BallScrewStabilizer:3 ↔ Nema23-StepperMotor:3
- Mate:403 (2 mm): Nema23-StepperMotor:3 ↔ MH2025-6.35x10mmCoupler:3
- Mate:404: BF12-BallScrewStabilizer2:3 ↔ SFU1605-BallScrew300mm:1
- Mate:405: BF12-BallScrewStabilizer2:3 ↔ SFU1605-BallScrew300mm:1
- Mate:406: BK12-BallScrewStabilizer:3 ↔ SFU1605-BallScrew300mm:1
- Mate:407 (2 mm): MH2025-6.35x10mmCoupler:3 ↔ SFU1605-BallScrew300mm:1
- Mate:408: 20x40x500mm-Extrusion2:2 ↔ RouterSpindle-65mm:1
- Mate:409 (14.505 mm): HGH20-LinearRailCarriage:10 ↔ DSG16H-BallScrewFixtureBlock:3
- Mate:410: HGH20-LinearRailCarriage:10 ↔ CNC-014-ZAxisSubMount1:1
- Mate:411: HGH20-LinearRailCarriage:10 ↔ CNC-014-ZAxisSubMount1:1
- Mate:412: HGH20-LinearRailCarriage:10 ↔ CNC-014-ZAxisSubMount1:1
- Mate:415: CNC-010-XAxisLimitSwitchMount:1 ↔ 90327A125-M5x10mm-LowProfileSCS:2
- Mate:416: CNC-010-XAxisLimitSwitchMount:1 ↔ 90327A125-M5x10mm-LowProfileSCS:1
- Flush:201: 90327A125-M5x10mm-LowProfileSCS:1 ↔ 90327A125-M5x10mm-LowProfileSCS:2
- Mate:420: CNC-010-XAxisLimitSwitchMount:1 ↔ 90327A125-M5x10mm-LowProfileSCS:2
- Mate:421: CNC-014-ZAxisSubMount1:1 ↔ 90327A125-M5x10mm-LowProfileSCS:8
- Mate:422: CNC-014-ZAxisSubMount1:1 ↔ 90327A125-M5x10mm-LowProfileSCS:7
- Mate:423: CNC-014-ZAxisSubMount1:1 ↔ 90327A125-M5x10mm-LowProfileSCS:6
- Mate:424: CNC-014-ZAxisSubMount1:1 ↔ 90327A125-M5x10mm-LowProfileSCS:5
- Mate:425: CNC-014-ZAxisSubMount1:1 ↔ 90327A125-M5x10mm-LowProfileSCS:5
- Flush:202: 90327A125-M5x10mm-LowProfileSCS:5 ↔ 90327A125-M5x10mm-LowProfileSCS:7
- Flush:203: 90327A125-M5x10mm-LowProfileSCS:7 ↔ 90327A125-M5x10mm-LowProfileSCS:8
- Flush:204: 90327A125-M5x10mm-LowProfileSCS:6 ↔ 90327A125-M5x10mm-LowProfileSCS:8
- Mate:426: CNC-014-ZAxisSubMount1:1 ↔ 90327A125-M5x10mm-LowProfileSCS:9
- Mate:427: CNC-014-ZAxisSubMount1:1 ↔ 90327A125-M5x10mm-LowProfileSCS:11
- Mate:428: CNC-014-ZAxisSubMount1:1 ↔ 90327A125-M5x10mm-LowProfileSCS:12
- Mate:429: CNC-014-ZAxisSubMount1:1 ↔ 90327A125-M5x10mm-LowProfileSCS:10
- Mate:430: CNC-014-ZAxisSubMount1:1 ↔ 90327A125-M5x10mm-LowProfileSCS:10
- Flush:205: 90327A125-M5x10mm-LowProfileSCS:10 ↔ 90327A125-M5x10mm-LowProfileSCS:11
- Flush:206: 90327A125-M5x10mm-LowProfileSCS:9 ↔ 90327A125-M5x10mm-LowProfileSCS:11
- Flush:207: 90327A125-M5x10mm-LowProfileSCS:9 ↔ 90327A125-M5x10mm-LowProfileSCS:12
- Mate:431: CNC-014-ZAxisSubMount1:1 ↔ 91290A231-M5x15mm:96
- Mate:432: CNC-014-ZAxisSubMount1:1 ↔ 91290A231-M5x15mm:96
- Mate:433: CNC-014-ZAxisSubMount1:1 ↔ 91290A231-M5x15mm:99
- Mate:434: CNC-014-ZAxisSubMount1:1 ↔ 91290A231-M5x15mm:98
- Mate:435: CNC-014-ZAxisSubMount1:1 ↔ 91290A231-M5x15mm:97
- Flush:208: 91290A231-M5x15mm:97 ↔ 91290A231-M5x15mm:99
- Flush:209: 91290A231-M5x15mm:97 ↔ 91290A231-M5x15mm:98
- Flush:210: 91290A231-M5x15mm:96 ↔ 91290A231-M5x15mm:98
- Mate:436: CNC-014-ZAxisSubMount1:1 ↔ 90327A125-M5x10mm-LowProfileSCS:13
- Mate:437: CNC-014-ZAxisSubMount1:1 ↔ 90327A125-M5x10mm-LowProfileSCS:13
- Mate:438: CNC-014-ZAxisSubMount1:1 ↔ 90327A125-M5x10mm-LowProfileSCS:14
- Flush:211: 90327A125-M5x10mm-LowProfileSCS:13 ↔ 90327A125-M5x10mm-LowProfileSCS:14
- Mate:439: CNC-014-ZAxisSubMount1:1 ↔ 90327A125-M5x10mm-LowProfileSCS:15
- Mate:440: CNC-014-ZAxisSubMount1:1 ↔ 90327A125-M5x10mm-LowProfileSCS:16
- Flush:212: 90327A125-M5x10mm-LowProfileSCS:15 ↔ 90327A125-M5x10mm-LowProfileSCS:16
- Flush:213: 90327A125-M5x10mm-LowProfileSCS:13 ↔ 90327A125-M5x10mm-LowProfileSCS:15